# Autodesk Inventor assembly: Interface-box
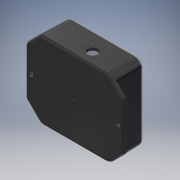
[picture p0: Inventor's stored thumbnail of the model, 180x180]
Saved by Autodesk Inventor 2018 (Build 220112000, 112)
## iProperties
Created: 2018-07-15
Part Number: Interface-box
Document SubType Name: Assembly
Designer: Tsche
Author: Tsche
## Documents named in this file (3)
- C:\Users\Tsche\Documents\MSE\MA\turtlebot_mods\Interface-box.iam
- C:\Users\Tsche\Documents\MSE\MA\turtlebot_mods\Interface-box.ipt
- C:\Users\Tsche\Documents\MSE\MA\turtlebot_mods\Interface-box_lid.ipt
## Components (2 placed, 2 different names)
1. Interface-box:1 — Mate:1, Mate:2, Mate:3
2. Interface-box_lid:1 — Mate:1, Mate:2, Mate:3
## Relationships (3: Mate 3)
- Mate:1: Interface-box:1 ↔ Interface-box_lid:1
- Mate:2: Interface-box:1 ↔ Interface-box_lid:1
- Mate:3: Interface-box:1 ↔ Interface-box_lid:1
